# Autodesk Inventor assembly: Middle Wheel Assembly
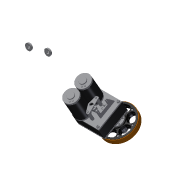
[picture p0: Inventor's stored thumbnail of the model, 180x180]
Saved by Autodesk Inventor 2014 SP1 (Build 180222100, 222)
## iProperties
Created: 2014-01-27
Part Number: Middle Wheel Assembly
Document SubType Name: Assembly
Designer: atslo_000
Author: atslo_000
## Documents named in this file (5)
- C:\Users\atslo_000\Desktop\2014 Robot V2\Chassis with Electrical Boards, Drive Train, and Battery\Middle Wheel Assembly\Middle Wheel Assembly.iam
- C:\Users\atslo_000\Desktop\2014 Robot V2\Chassis with Electrical Boards, Drive Train, and Battery\Middle Wheel Assembly\super-shifter-asm-penumatic-hex-long\super-shifter-asm-penumatic-hex-long.iam
- C:\Users\atslo_000\Desktop\2014 Robot V2\Chassis with Electrical Boards, Drive Train, and Battery\Middle Wheel Assembly\fr8zz-hex.ipt
- C:\Users\atslo_000\Desktop\2014 Robot V2\Chassis with Electrical Boards, Drive Train, and Battery\Middle Wheel Assembly\500_hex_hub.ipt
- C:\Users\atslo_000\Desktop\2014 Robot V2\Chassis with Electrical Boards, Drive Train, and Battery\Middle Wheel Assembly\6Plaction-asm\6Plaction-asm.iam
## Components (7 placed, 4 different names)
1. super-shifter-asm-penumatic-hex-long:1 [sub-assembly] — Mate:1, Mate:2, Flush:1, Mate:3, Mate:4, Mate:6, Mate:7
2. fr8zz-hex:1
3. fr8zz-hex:2
4. fr8zz-hex:3 — Mate:1, Mate:2, Flush:1, Mate:5
5. 500_hex_hub:1 — Mate:3, Mate:4, Mate:5, Mate:9
6. 6Plaction-asm:1 [sub-assembly] — Mate:6, Mate:8, Mate:9
7. 500_hex_hub:2 — Mate:7, Mate:8
## Relationships (10: Mate 9, Flush 1)
- Mate:1: super-shifter-asm-penumatic-hex-long:1 ↔ fr8zz-hex:3
- Mate:2: super-shifter-asm-penumatic-hex-long:1 ↔ fr8zz-hex:3
- Flush:1 (-1.7272 mm): super-shifter-asm-penumatic-hex-long:1 ↔ fr8zz-hex:3
- Mate:3: super-shifter-asm-penumatic-hex-long:1 ↔ 500_hex_hub:1
- Mate:4: super-shifter-asm-penumatic-hex-long:1 ↔ 500_hex_hub:1
- Mate:5 (16.1544 mm): fr8zz-hex:3 ↔ 500_hex_hub:1
- Mate:6: super-shifter-asm-penumatic-hex-long:1 ↔ 6Plaction-asm:1
- Mate:7: super-shifter-asm-penumatic-hex-long:1 ↔ 500_hex_hub:2
- Mate:8: 6Plaction-asm:1 ↔ 500_hex_hub:2
- Mate:9: 500_hex_hub:1 ↔ 6Plaction-asm:1
